# Autodesk Inventor assembly: nozzle
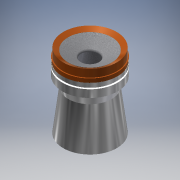
[picture p0: Inventor's stored thumbnail of the model, 180x180]
Saved by Autodesk Inventor 2017 SP1 (Build 210196100, 196)
## iProperties
Created: 2016-10-24
Part Number: nozzle
Document SubType Name: Assembly
Designer: cflannery
Author: cflannery
## Documents named in this file (6)
- D:\Triton_Rocket_Club\Propulsion\Users\cflannery\Temporary_Work\Nozzle_designSpace\nozzle.iam
- D:\Triton_Rocket_Club\Propulsion\Users\cflannery\Temporary_Work\Nozzle_designSpace\aluminum_carrier.ipt
- D:\Triton_Rocket_Club\Propulsion\Users\cflannery\Temporary_Work\Nozzle_designSpace\aluminum_retainer.ipt
- D:\Triton_Rocket_Club\Propulsion\Users\cflannery\Temporary_Work\Nozzle_designSpace\graphite.ipt
- D:\Triton_Rocket_Club\Propulsion\Users\cflannery\Temporary_Work\Nozzle_designSpace\phenolic_bottom.ipt
- D:\Triton_Rocket_Club\Propulsion\Users\cflannery\Temporary_Work\Nozzle_designSpace\phenolic_top.ipt
## Components (5 placed, 5 different names)
1. aluminum_carrier:1 — Mate:3, Mate:6, Mate:7
2. aluminum_retainer:1 — Mate:2, Mate:7
3. graphite:1 — Mate:1, Mate:2, Mate:3, Mate:4, Mate:5
4. phenolic_bottom:1 — Mate:1, Mate:8
5. phenolic_top:1 — Mate:4, Mate:5, Mate:6, Mate:8
## Relationships (8: Mate 8)
- Mate:1: graphite:1 ↔ phenolic_bottom:1
- Mate:2: aluminum_retainer:1 ↔ graphite:1
- Mate:3: aluminum_carrier:1 ↔ graphite:1
- Mate:4: graphite:1 ↔ phenolic_top:1
- Mate:5: graphite:1 ↔ phenolic_top:1
- Mate:6: aluminum_carrier:1 ↔ phenolic_top:1
- Mate:7: aluminum_carrier:1 ↔ aluminum_retainer:1
- Mate:8: phenolic_bottom:1 ↔ phenolic_top:1
